# Autodesk Inventor assembly: Upper_Arm_v2_Assembly
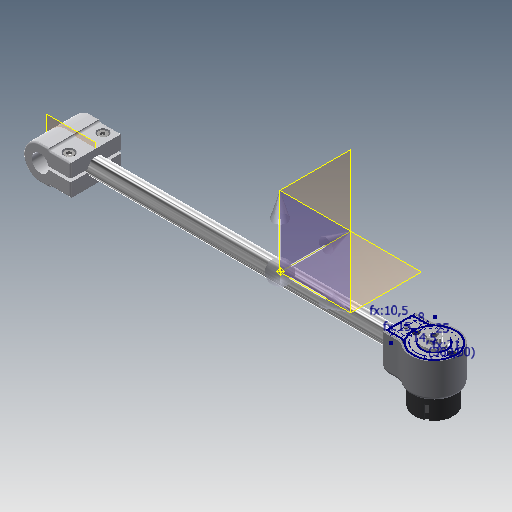
[picture p0: Inventor's stored thumbnail of the model, 512x512]
Saved by Autodesk Inventor 2021.4 (Build 254397000, 397)
## iProperties
Created: 2022-07-06
Part Number: Upper_Arm_v2_Assembly
Material: Generisch
Document SubType Name: Assembly
Designer: alexw
Mass: 56.2336 g
Surface Area: 309.167 cm^2
Volume: 28.4426 cm^3
Density: 1.97709 g/cm^3
Author: alexw
## Documents named in this file (12)
- C:\Users\alexw\Documents\Inventor\Projects\03_CurrentProjects\MasterThesis\TrainingConsol_220422\Workgroups\Workgroup\Upper_Arm_v2_Assembly.iam
- C:\Users\alexw\Documents\Inventor\Projects\03_CurrentProjects\MasterThesis\TrainingConsol_220422\Workgroups\Workgroup\UpperArm_Yawn_Fixture.ipt
- C:\Users\alexw\Documents\Inventor\Projects\03_CurrentProjects\MasterThesis\TrainingConsol_220422\Workgroups\Workgroup\Upper_Arm_Shaft.ipt
- C:\Users\alexw\Documents\Inventor\Projects\03_CurrentProjects\MasterThesis\TrainingConsol_220422\Workgroups\Workgroup\ContentCenter\en-US\ISO 4762(2)\ISO 4762 - M3 x 8ISO.ipt
- C:\Users\alexw\Documents\Inventor\Projects\03_CurrentProjects\MasterThesis\TrainingConsol_220422\Workgroups\Workgroup\Downloads\W 6178\SKF_W 617_8.iam
- C:\Users\alexw\Documents\Inventor\Projects\03_CurrentProjects\MasterThesis\TrainingConsol_220422\Workgroups\Workgroup\Lower_Arm_Cover_v2.ipt
- C:\Users\alexw\Documents\Inventor\Projects\03_CurrentProjects\MasterThesis\TrainingConsol_220422\Workgroups\Workgroup\Magnetic Encoder.ipt
- C:\Users\alexw\Documents\Inventor\Projects\03_CurrentProjects\MasterThesis\TrainingConsol_220422\Workgroups\Workgroup\UpperLowerArm_JointShaft.ipt
- C:\Users\alexw\Documents\Inventor\Projects\03_CurrentProjects\MasterThesis\TrainingConsol_220422\Workgroups\Workgroup\Downloads\DIN471_a_8_unstressed.ipt
- C:\Users\alexw\Documents\Inventor\Projects\03_CurrentProjects\MasterThesis\TrainingConsol_220422\Workgroups\Workgroup\Lower_Arm_v4_printversion.ipt
- C:\Users\alexw\Documents\Inventor\Projects\03_CurrentProjects\MasterThesis\TrainingConsol_220422\Workgroups\Workgroup\Downloads\din_913-m3x5-45h.ipt
- C:\Users\alexw\Documents\Inventor\Projects\03_CurrentProjects\MasterThesis\TrainingConsol_220422\Workgroups\Workgroup\ContentCenter\en-US\ISO 7046-1 H(1)\ISO 7046-1 - M2 x 10_ - 4.8 - H - ISO.ipt
## Components (14 placed, 11 different names)
1. UpperArm_Yawn_Fixture:1 — Flush:1, Flush:2, Flush:3, Mate:1, Tangent:1, Mate:2, Mate:3, Mate:4, Mate:5, Angle:1, Angle:2
2. Upper_Arm_Shaft:1 — Mate:1, Tangent:1, Mate:42, Flush:4, Tangent:2
3. ISO 4762 M3 x 8:1 — Mate:2, Mate:3
4. ISO 4762 M3 x 8:2 — Mate:4, Mate:5
5. Lower_Arm_v4_printversion:1 — Mate:42, Flush:4, Mate:44, Mate:45, Angle:2, Mate:46, Mate:47, Mate:48, Mate:49, Mate:50
6. SKF_W 617_8:1 [sub-assembly] — Mate:37, Mate:38
7. SKF_W 617_8:2 [sub-assembly] — Mate:37, Mate:39, Mate:43, Mate:44, Mate:45
8. Lower_Arm_Cover_v2:1 — Mate:19, Mate:20, Mate:21, Angle:1, Mate:46, Mate:47
9. Magnetic Encoder:1 — Mate:19, Mate:20, Mate:21
10. UpperLowerArm_JointShaft:1 — Mate:38, Mate:39, Mate:40, Mate:41, Mate:43
11. DIN471_a_8_unstressed:1 — Mate:40, Mate:41
12. din_913-m3x5-45h:1 — Mate:48, Tangent:2
13. ISO 7046-1 H M2 x 10 - 4.8 - H:1 — Mate:49
14. ISO 7046-1 H M2 x 10 - 4.8 - H:2 — Mate:50
## Relationships (30: Mate 22, Flush 4, Tangent 2, Angle 2)
- Flush:1: UpperArm_Yawn_Fixture:1
- Flush:2: UpperArm_Yawn_Fixture:1
- Flush:3: UpperArm_Yawn_Fixture:1
- Mate:1: UpperArm_Yawn_Fixture:1 ↔ Upper_Arm_Shaft:1
- Tangent:1: UpperArm_Yawn_Fixture:1 ↔ Upper_Arm_Shaft:1
- Mate:2: UpperArm_Yawn_Fixture:1 ↔ ISO 4762 M3 x 8:1
- Mate:3: UpperArm_Yawn_Fixture:1 ↔ ISO 4762 M3 x 8:1
- Mate:4: UpperArm_Yawn_Fixture:1 ↔ ISO 4762 M3 x 8:2
- Mate:5: UpperArm_Yawn_Fixture:1 ↔ ISO 4762 M3 x 8:2
- Mate:19: Lower_Arm_Cover_v2:1 ↔ Magnetic Encoder:1
- Mate:20: Lower_Arm_Cover_v2:1 ↔ Magnetic Encoder:1
- Mate:21: Lower_Arm_Cover_v2:1 ↔ Magnetic Encoder:1
- Angle:1 (0 deg): UpperArm_Yawn_Fixture:1 ↔ Lower_Arm_Cover_v2:1
- Mate:37: SKF_W 617_8:1 ↔ SKF_W 617_8:2
- Mate:38: SKF_W 617_8:1 ↔ UpperLowerArm_JointShaft:1
- Mate:39: SKF_W 617_8:2 ↔ UpperLowerArm_JointShaft:1
- Mate:40: UpperLowerArm_JointShaft:1 ↔ DIN471_a_8_unstressed:1
- Mate:41: UpperLowerArm_JointShaft:1 ↔ DIN471_a_8_unstressed:1
- Mate:42: Upper_Arm_Shaft:1 ↔ Lower_Arm_v4_printversion:1
- Flush:4: Upper_Arm_Shaft:1 ↔ Lower_Arm_v4_printversion:1
- Mate:43: SKF_W 617_8:2 ↔ UpperLowerArm_JointShaft:1
- Mate:44: Lower_Arm_v4_printversion:1 ↔ SKF_W 617_8:2
- Mate:45: Lower_Arm_v4_printversion:1 ↔ SKF_W 617_8:2
- Angle:2 (0 deg): UpperArm_Yawn_Fixture:1 ↔ Lower_Arm_v4_printversion:1
- Mate:46: Lower_Arm_v4_printversion:1 ↔ Lower_Arm_Cover_v2:1
- Mate:47: Lower_Arm_v4_printversion:1 ↔ Lower_Arm_Cover_v2:1
- Mate:48: Lower_Arm_v4_printversion:1 ↔ din_913-m3x5-45h:1
- Tangent:2: Upper_Arm_Shaft:1 ↔ din_913-m3x5-45h:1
- Mate:49: Lower_Arm_v4_printversion:1 ↔ ISO 7046-1 H M2 x 10 - 4.8 - H:1
- Mate:50: Lower_Arm_v4_printversion:1 ↔ ISO 7046-1 H M2 x 10 - 4.8 - H:2
